# Autodesk Inventor assembly: Assembly2
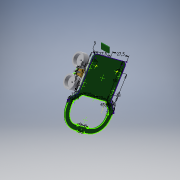
[picture p0: Inventor's stored thumbnail of the model, 180x180]
Saved by Autodesk Inventor 2016 (Build 200138000, 138)
## iProperties
Created: 2017-05-26
Part Number: Assembly2
Material: Ogólny
Document SubType Name: Assembly
Designer: Karol
Author: Karol
## Documents named in this file (11)
- D:\Git\MicromouseDixi\hardware\models\Dixi.iam
- D:\Git\MicromouseDixi\hardware\models\wheel.ipt
- D:\Git\MicromouseDixi\hardware\models\togh.ipt
- D:\Git\MicromouseDixi\hardware\models\bolt.ipt
- D:\Git\MicromouseDixi\hardware\models\magnet.ipt
- D:\Git\MicromouseDixi\hardware\models\mainpcb.ipt
- D:\Git\MicromouseDixi\hardware\models\motor.ipt
- D:\ele\MicroMouse\v2\hardware\models\top_mount.ipt
- D:\ele\MicroMouse\v2\hardware\models\enc_pcb.ipt
- D:\Git\MicromouseDixi\hardware\models\XSM_0203_03_1.ipt
- D:\Git\MicromouseDixi\hardware\models\XFM_020406_03_233.ipt
## Components (14 placed, 10 different names)
1. mainpcb:1 — Rigid:38
2. bolt:3 — Rigid:15, Rigid:45
3. bolt:4 — Rigid:14, Rigid:46
4. wheel:3 — Rigid:15
5. wheel:4 — Rigid:14
6. magnet:4
7. togh:2 — Rigid:38, Rigid:39, Rigid:40, Rigid:41, Rigid:44
8. motor:1 — Rigid:39
9. top_mount:1 — Rigid:40
10. enc_pcb:1
11. XSM_0203_03_1:1 — Rigid:42, Rigid:45
12. XFM_020406_03_233:1 — Rigid:41, Rigid:42
13. XSM_0203_03_1:2 — Rigid:46
14. XFM_020406_03_233:2 — Rigid:44
## Relationships (12: WeldJoint 12)
- Rigid:14 [WeldJoint] (-1.8 mm): bolt:4 ↔ wheel:4
- Rigid:15 [WeldJoint] (-1.8 mm): bolt:3 ↔ wheel:3
- [WeldJoint]: bolt:4 ↔ magnet:4
- Rigid:38 [WeldJoint]: mainpcb:1 ↔ togh:2
- Rigid:39 [WeldJoint]: togh:2 ↔ motor:1
- Rigid:40 [WeldJoint]: togh:2 ↔ top_mount:1
- Rigid:41 [WeldJoint] (-1.5 mm): togh:2 ↔ XFM_020406_03_233:1
- Rigid:42 [WeldJoint]: XSM_0203_03_1:1 ↔ XFM_020406_03_233:1
- [WeldJoint]: XSM_0203_03_1:2 ↔ XFM_020406_03_233:2
- Rigid:44 [WeldJoint] (1 mm): togh:2 ↔ XFM_020406_03_233:2
- Rigid:45 [WeldJoint]: bolt:3 ↔ XSM_0203_03_1:1
- Rigid:46 [WeldJoint]: bolt:4 ↔ XSM_0203_03_1:2
## Named parameters: d111_d4 = -1.8 mm, d112_d5 = 0.127925 deg, d113_d6 = -1.8 mm, d114_d7 = -6.839272 deg, d117_d14 = 0 mm, d118_d15 = 2.56641 deg, d234_d233 = 0 mm
